# Autodesk Inventor assembly: 5 Barras Version 0
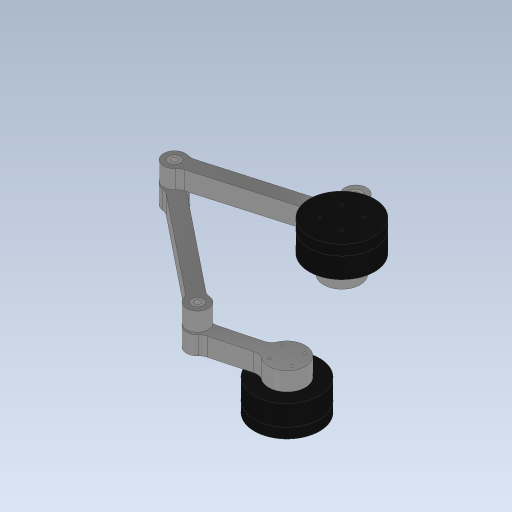
[picture p0: Inventor's stored thumbnail of the model, 512x512]
Saved by Autodesk Inventor 2024.2 (Build 282272000, 272)
## iProperties
Created: 2025-02-06
Part Number: 5 Barras Version 0
Document SubType Name: Assembly
Designer: jp.reyesf
Author: jp.reyesf
## Documents named in this file (13)
- C:\Users\jp.reyesf\Desktop\Master-Thesis\five_bar\assets\CAD\Robot\5 Barras Version 0.iam
- C:\Users\jp.reyesf\Desktop\Master-Thesis\five_bar\assets\CAD\Robot\Proximal Link 1.ipt
- C:\Users\jp.reyesf\Desktop\Master-Thesis\five_bar\assets\CAD\Robot\Distal Link 1.ipt
- C:\Users\jp.reyesf\Desktop\Master-Thesis\five_bar\assets\CAD\Robot\Distal Link 2.ipt
- C:\Users\jp.reyesf\Desktop\Master-Thesis\five_bar\assets\CAD\Robot\Proximal Link 2.ipt
- C:\Users\jp.reyesf\Desktop\Master-Thesis\five_bar\assets\CAD\Robot\Spacer.ipt
- C:\Users\jp.reyesf\Desktop\Master-Thesis\five_bar\assets\CAD\Robot\Bearing.ipt
- C:\Users\jp.reyesf\Desktop\Master-Thesis\five_bar\assets\CAD\Robot\Motor 1 Stator.ipt
- C:\Users\jp.reyesf\Desktop\Master-Thesis\five_bar\assets\CAD\Robot\Motor 1 Rotor.ipt
- C:\Users\jp.reyesf\Desktop\Master-Thesis\five_bar\assets\CAD\Robot\Motor 2 Stator.ipt
- C:\Users\jp.reyesf\Desktop\Master-Thesis\five_bar\assets\CAD\Robot\Motor 2 Rotor.ipt
- C:\Users\jp.reyesf\Desktop\Master-Thesis\five_bar\assets\CAD\Robot\separator.ipt
- C:\Users\jp.reyesf\Desktop\Master-Thesis\five_bar\assets\CAD\Robot\rod.ipt
## Components (32 placed, 12 different names)
1. Proximal Link 1:1 — Mate:3, Mate:4, Mate:5, Mate:30, Flush:1, Mate:36, Mate:37, Mate:39, Mate:52
2. Distal Link 1:1 — Mate:31, Mate:32, Flush:2, Flush:3, Mate:38, Mate:39, Mate:40, Mate:41, Mate:43, Flush:7
3. Distal Link 2:1 — Mate:33, Mate:34, Flush:4, Flush:5, Mate:42, Mate:43, Mate:44, Mate:45, Mate:47, Flush:8, Mate:53
4. Proximal Link 2:1 — Mate:35, Flush:6, Mate:46, Mate:47, Mate:48, Mate:49, Flush:9, Mate:54
5. Spacer:1 — Mate:6, Mate:7, Mate:8, Mate:9, Mate:33
6. Bearing:1 — Mate:6, Mate:8
7. Motor 1 Stator:1 — Mate:1, Mate:2
8. Motor 1 Rotor:1 — Mate:1, Mate:2, Mate:3, Mate:4, Mate:5
9. Motor 2 Stator:1 — Mate:50, Mate:51
10. Motor 2 Rotor:1 — Mate:48, Mate:49, Mate:50, Mate:51
11. separator:1 — Mate:36, Mate:37, Mate:38
12. separator:2 — Mate:44, Mate:45, Mate:46
13. separator:3 — Mate:40, Mate:41, Mate:42
14. Bearing:3 — Mate:7, Mate:9, Flush:4
15. Spacer:2 — Mate:35
16. Bearing:4 — Flush:6
17. Bearing:5
18. Spacer:3 — Mate:34
19. Bearing:6
20. Bearing:7 — Flush:5
21. Spacer:4 — Mate:30
22. Bearing:8 — Flush:1
23. Bearing:9
24. Spacer:5 — Mate:32
25. Bearing:10 — Flush:2
26. Bearing:11
27. Spacer:6 — Mate:31
28. Bearing:12 — Flush:3
29. Bearing:13
30. rod:1 — Flush:7, Mate:52
31. rod:2 — Flush:8, Mate:53
32. rod:3 — Flush:9, Mate:54
## Relationships (63: Mate 54, Flush 9)
- Mate:1: Motor 1 Stator:1 ↔ Motor 1 Rotor:1
- Mate:2: Motor 1 Stator:1 ↔ Motor 1 Rotor:1
- Mate:3: Proximal Link 1:1 ↔ Motor 1 Rotor:1
- Mate:4: Proximal Link 1:1 ↔ Motor 1 Rotor:1
- Mate:5: Proximal Link 1:1 ↔ Motor 1 Rotor:1
- Mate:6: Spacer:1 ↔ Bearing:1
- Mate:7: Spacer:1 ↔ Bearing:3
- Mate:8: Spacer:1 ↔ Bearing:1
- Mate:9: Spacer:1 ↔ Bearing:3
- [Mate]: Spacer:2 ↔ Bearing:4
- [Mate]: Spacer:2 ↔ Bearing:5
- [Mate]: Spacer:2 ↔ Bearing:4
- [Mate]: Spacer:2 ↔ Bearing:5
- [Mate]: Spacer:3 ↔ Bearing:6
- [Mate]: Spacer:3 ↔ Bearing:7
- [Mate]: Spacer:3 ↔ Bearing:6
- [Mate]: Spacer:3 ↔ Bearing:7
- [Mate]: Spacer:4 ↔ Bearing:8
- [Mate]: Spacer:4 ↔ Bearing:9
- [Mate]: Spacer:4 ↔ Bearing:8
- [Mate]: Spacer:4 ↔ Bearing:9
- [Mate]: Spacer:5 ↔ Bearing:10
- [Mate]: Spacer:5 ↔ Bearing:11
- [Mate]: Spacer:5 ↔ Bearing:10
- [Mate]: Spacer:5 ↔ Bearing:11
- [Mate]: Spacer:6 ↔ Bearing:12
- [Mate]: Spacer:6 ↔ Bearing:13
- [Mate]: Spacer:6 ↔ Bearing:12
- [Mate]: Spacer:6 ↔ Bearing:13
- Mate:30: Proximal Link 1:1 ↔ Spacer:4
- Flush:1: Proximal Link 1:1 ↔ Bearing:8
- Mate:31: Distal Link 1:1 ↔ Spacer:6
- Mate:32: Distal Link 1:1 ↔ Spacer:5
- Flush:2: Distal Link 1:1 ↔ Bearing:10
- Flush:3: Distal Link 1:1 ↔ Bearing:12
- Mate:33: Distal Link 2:1 ↔ Spacer:1
- Mate:34: Distal Link 2:1 ↔ Spacer:3
- Mate:35: Proximal Link 2:1 ↔ Spacer:2
- Flush:4: Distal Link 2:1 ↔ Bearing:3
- Flush:5: Distal Link 2:1 ↔ Bearing:7
- Flush:6: Proximal Link 2:1 ↔ Bearing:4
- Mate:36: Proximal Link 1:1 ↔ separator:1
- Mate:37: Proximal Link 1:1 ↔ separator:1
- Mate:38: Distal Link 1:1 ↔ separator:1
- Mate:39: Proximal Link 1:1 ↔ Distal Link 1:1
- Mate:40: Distal Link 1:1 ↔ separator:3
- Mate:41: Distal Link 1:1 ↔ separator:3
- Mate:42: Distal Link 2:1 ↔ separator:3
- Mate:43: Distal Link 1:1 ↔ Distal Link 2:1
- Mate:44: Distal Link 2:1 ↔ separator:2
- Mate:45: Distal Link 2:1 ↔ separator:2
- Mate:46: Proximal Link 2:1 ↔ separator:2
- Mate:47: Distal Link 2:1 ↔ Proximal Link 2:1
- Mate:48: Proximal Link 2:1 ↔ Motor 2 Rotor:1
- Mate:49: Proximal Link 2:1 ↔ Motor 2 Rotor:1
- Mate:50: Motor 2 Stator:1 ↔ Motor 2 Rotor:1
- Mate:51: Motor 2 Stator:1 ↔ Motor 2 Rotor:1
- Flush:7: Distal Link 1:1 ↔ rod:1
- Flush:8: Distal Link 2:1 ↔ rod:2
- Flush:9: Proximal Link 2:1 ↔ rod:3
- Mate:52: Proximal Link 1:1 ↔ rod:1
- Mate:53: Distal Link 2:1 ↔ rod:2
- Mate:54: Proximal Link 2:1 ↔ rod:3
## Named parameters: d18_d14 = 0 mm, d19_d15 = 0 mm, d20_d16 = 0 mm, d21_d17 = 0 mm, d22_d14 = 0 mm, d23_d15 = 0 mm, d24_d16 = 0 mm, d25_d17 = 0 mm, d26_d14 = 0 mm, d27_d15 = 0 mm, d28_d16 = 0 mm, d29_d17 = 0 mm, d30_d14 = 0 mm, d31_d15 = 0 mm, d32_d16 = 0 mm, d33_d17 = 0 mm, d34_d14 = 0 mm, d35_d15 = 0 mm, d36_d16 = 0 mm, d37_d17 = 0 mm
